# Autodesk Inventor assembly: DeriveAssem
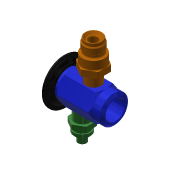
[picture p0: Inventor's stored thumbnail of the model, 180x180]
Saved by Autodesk Inventor 2022 (Build 260148000, 148)
## iProperties
Created: 2009-04-14
Part Number: DeriveAssem
Document SubType Name: Assembly
Designer: User
Author: User
## Documents named in this file (5)
- C:\Autodesk Inventor 2022 Advanced Assembly Modeling Practice Files\Derive Assem.iam
- C:\Autodesk Inventor 2022 Advanced Assembly Modeling Practice Files\102650.ipt
- C:\Autodesk Inventor 2022 Advanced Assembly Modeling Practice Files\102651.ipt
- C:\Autodesk Inventor 2022 Advanced Assembly Modeling Practice Files\102652.ipt
- C:\Autodesk Inventor 2022 Advanced Assembly Modeling Practice Files\102653.ipt
## Components (4 placed, 4 different names)
1. 102650:1 — Insert:1
2. 102652:2 — Insert:2
3. 102653:3 — Insert:1, Insert:2, Insert:3
4. 102651:4 — Insert:3
## Relationships (3: Insert 3)
- Insert:1: 102650:1 ↔ 102653:3
- Insert:2: 102652:2 ↔ 102653:3
- Insert:3: 102653:3 ↔ 102651:4
